# Autodesk Inventor assembly: caenDT5702PinBreakout
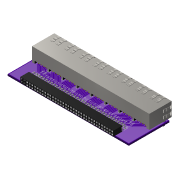
[picture p0: Inventor's stored thumbnail of the model, 180x180]
Saved by Autodesk Inventor 2018 (Build 220112000, 112)
## iProperties
Created: 2017-06-08
Part Number: caenDT5702PinBreakout
Document SubType Name: Assembly
Designer: sawaiz
Author: sawaiz
## Documents named in this file (4)
- C:\Users\sawaiz\OneDrive\projects\sPHENIXTileTest\caenDT5702PinBreakout\cad\caenDT5702PinBreakout.iam
- C:\Users\sawaiz\OneDrive\projects\sPHENIXTileTest\caenDT5702PinBreakout\cad\caenDT5702PinBreakout.ipt
- C:\Users\sawaiz\OneDrive\projects\sPHENIXTileTest\caenDT5702PinBreakout\cad\SS-668808S-A-PG4-AC.ipt
- C:\Users\sawaiz\OneDrive\projects\sPHENIXTileTest\caenDT5702PinBreakout\cad\_ _ _C362LJBN-RC.ipt
## Components (3 placed, 3 different names)
1. caenDT5702PinBreakout:1 — Mate:1, Mate:2, Angle:1, Mate:3, Angle:2
2. SS-668808S-A-PG4-AC:1 — Mate:1, Mate:2, Angle:1
3. _ _ _C362LJBN-RC:1 — Mate:3, Angle:2
## Relationships (5: Mate 3, Angle 2)
- Mate:1: caenDT5702PinBreakout:1 ↔ SS-668808S-A-PG4-AC:1
- Mate:2: caenDT5702PinBreakout:1 ↔ SS-668808S-A-PG4-AC:1
- Angle:1 (0 deg): caenDT5702PinBreakout:1 ↔ SS-668808S-A-PG4-AC:1
- Mate:3: caenDT5702PinBreakout:1 ↔ _ _ _C362LJBN-RC:1
- Angle:2 (0 deg): caenDT5702PinBreakout:1 ↔ _ _ _C362LJBN-RC:1
